# Autodesk Inventor assembly: Ensamblaje1
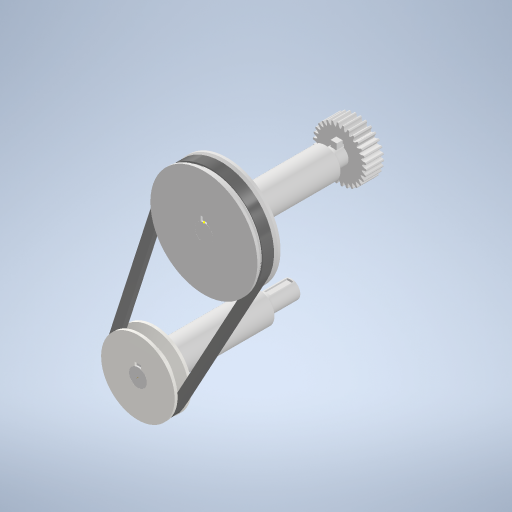
[picture p0: Inventor's stored thumbnail of the model, 512x512]
Saved by Autodesk Inventor 2024 (Build 280153000, 153)
## iProperties
Created: 2024-03-07
Part Number: Ensamblaje1
Document SubType Name: Assembly
Designer: joseo
Author: joseo
## Documents named in this file (6)
- C:\Users\joseo\OneDrive - Universidad Rafael Landivar\Documentos\DINAMICA\Ensamblaje1.iam
- C:\Users\joseo\OneDrive - Universidad Rafael Landivar\Documentos\DINAMICA\POLEA.ipt
- C:\Users\joseo\OneDrive - Universidad Rafael Landivar\Documentos\DINAMICA\EJE_CUÑEROS.ipt
- C:\Users\joseo\OneDrive - Universidad Rafael Landivar\Documentos\DINAMICA\ENGRANE.ipt
- C:\Users\joseo\OneDrive - Universidad Rafael Landivar\Documentos\DINAMICA\CUÑA.ipt
- C:\Users\joseo\OneDrive - Universidad Rafael Landivar\Documentos\DINAMICA\Ensamblaje1\Design Accelerator\Transmisión de correa trapezoidal1.iam
## Components (8 placed, 5 different names)
1. CUÑA:1 — Plana:1, Coincidencia:3
2. CUÑA:2 — Cilíndrica:3, Coincidencia:1, Coincidencia:2
3. ENGRANE:1 — Cilíndrica:2, Nivelación:2
4. EJE_CUÑEROS:1 — Cilíndrica:1, Nivelación:1, Cilíndrica:2, Nivelación:2, Cilíndrica:3, Coincidencia:1, Coincidencia:2, Plana:1, Coincidencia:3
5. POLEA:1 — Cilíndrica:1, Nivelación:1
6. Transmisión de correa trapezoidal:1 [sub-assembly] — Cilíndrica:4, Nivelación:3
7. EJE_CUÑEROS:2 — Cilíndrica:4, Nivelación:3, Rígido:1, Coincidencia:4
8. CUÑA:3 — Rígido:1, Coincidencia:4
## Relationships (13: CylindricalJoint 4, Mate 4, Flush 3, PlanarJoint 1, WeldJoint 1)
- Cilíndrica:1 [CylindricalJoint]: EJE_CUÑEROS:1 ↔ POLEA:1
- Nivelación:1 [Flush]: EJE_CUÑEROS:1 ↔ POLEA:1
- Cilíndrica:2 [CylindricalJoint]: ENGRANE:1 ↔ EJE_CUÑEROS:1
- Nivelación:2 [Flush]: ENGRANE:1 ↔ EJE_CUÑEROS:1
- Cilíndrica:3 [CylindricalJoint]: CUÑA:2 ↔ EJE_CUÑEROS:1
- Coincidencia:1 [Mate]: CUÑA:2 ↔ EJE_CUÑEROS:1
- Coincidencia:2 [Mate]: CUÑA:2 ↔ EJE_CUÑEROS:1
- Plana:1: CUÑA:1 ↔ EJE_CUÑEROS:1
- Coincidencia:3 [Mate]: CUÑA:1 ↔ EJE_CUÑEROS:1
- Cilíndrica:4 [CylindricalJoint]: Transmisión de correa trapezoidal:1 ↔ EJE_CUÑEROS:2
- Nivelación:3 [Flush]: Transmisión de correa trapezoidal:1 ↔ EJE_CUÑEROS:2
- Rígido:1 [WeldJoint]: EJE_CUÑEROS:2 ↔ CUÑA:3
- Coincidencia:4 [Mate]: EJE_CUÑEROS:2 ↔ CUÑA:3
